# Autodesk Inventor assembly: Assemblage
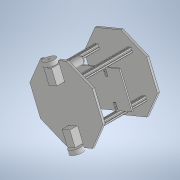
[picture p0: Inventor's stored thumbnail of the model, 180x180]
Saved by Autodesk Inventor 2020 (Build 240168000, 168)
## iProperties
Created: 2019-11-28
Part Number: Assemblage
Document SubType Name: Assembly
Designer: erwan
Author: erwan
## Documents named in this file (7)
- C:\Users\erwan\Desktop\Eirbot\Coupe robotique\Maquette robot\Assemblage.iam
- C:\Users\erwan\Desktop\Eirbot\Coupe robotique\Maquette robot\Pièces\Support bas.ipt
- C:\Users\erwan\Desktop\Eirbot\Coupe robotique\Maquette robot\Pièces\Profilé.ipt
- C:\Users\erwan\Desktop\Eirbot\Coupe robotique\Maquette robot\Pièces\Etage.ipt
- C:\Users\erwan\Desktop\Eirbot\Coupe robotique\Maquette robot\Pièces\Support haut.ipt
- C:\Users\erwan\Desktop\Eirbot\Coupe robotique\Maquette robot\Pièces\Equerre.ipt
- C:\Users\erwan\Desktop\Eirbot\Coupe robotique\Maquette robot\Pièces\Bloc-moteur.ipt
## Components (13 placed, 6 different names)
1. Support bas:1 — Placage:5, Affleurement:1, Affleurement:2, Placage:6, Affleurement:3, Affleurement:4, Placage:7, Placage:8, Placage:9, Placage:10, Affleurement:5, Affleurement:6, Affleurement:7, Affleurement:8, Placage:27, Placage:28, Affleurement:9, Placage:29, Placage:30, Affleurement:10
2. Etage:1 — Placage:5, Affleurement:1, Affleurement:2, Placage:13, Placage:14, Placage:17, Placage:18, Placage:21, Placage:22, Placage:25, Placage:26
3. Support haut:1 — Placage:6, Affleurement:3, Affleurement:4
4. Profilé:1 — Placage:10, Placage:23, Placage:24, Affleurement:8
5. Profilé:2 — Placage:9, Placage:15, Placage:16, Affleurement:6
6. Profilé:3 — Placage:8, Placage:11, Placage:12, Affleurement:5
7. Profilé:4 — Placage:7, Placage:19, Placage:20, Affleurement:7
8. Equerre:1 — Placage:11, Placage:12, Placage:13, Placage:14
9. Equerre:2 — Placage:15, Placage:16, Placage:17, Placage:18
10. Equerre:3 — Placage:19, Placage:20, Placage:21, Placage:22
11. Equerre:4 — Placage:23, Placage:24, Placage:25, Placage:26
12. Bloc-moteur:1 — Placage:29, Placage:30, Affleurement:10
13. Bloc-moteur:2 — Placage:27, Placage:28, Affleurement:9
## Relationships (36: Mate 26, Flush 10)
- Placage:5 [Mate] (125 mm): Support bas:1 ↔ Etage:1
- Affleurement:1 [Flush] (1.5 mm): Support bas:1 ↔ Etage:1
- Affleurement:2 [Flush] (1.5 mm): Support bas:1 ↔ Etage:1
- Placage:6 [Mate] (250 mm): Support bas:1 ↔ Support haut:1
- Affleurement:3 [Flush]: Support bas:1 ↔ Support haut:1
- Affleurement:4 [Flush]: Support bas:1 ↔ Support haut:1
- Placage:7 [Mate]: Support bas:1 ↔ Profilé:4
- Placage:8 [Mate]: Support bas:1 ↔ Profilé:3
- Placage:9 [Mate]: Support bas:1 ↔ Profilé:2
- Placage:10 [Mate]: Support bas:1 ↔ Profilé:1
- Placage:11 [Mate]: Profilé:3 ↔ Equerre:1
- Placage:12 [Mate]: Profilé:3 ↔ Equerre:1
- Placage:13 [Mate]: Etage:1 ↔ Equerre:1
- Placage:14 [Mate]: Etage:1 ↔ Equerre:1
- Placage:15 [Mate]: Profilé:2 ↔ Equerre:2
- Placage:16 [Mate]: Profilé:2 ↔ Equerre:2
- Placage:17 [Mate]: Etage:1 ↔ Equerre:2
- Placage:18 [Mate]: Etage:1 ↔ Equerre:2
- Placage:19 [Mate]: Profilé:4 ↔ Equerre:3
- Placage:20 [Mate]: Profilé:4 ↔ Equerre:3
- Placage:21 [Mate]: Etage:1 ↔ Equerre:3
- Placage:22 [Mate]: Etage:1 ↔ Equerre:3
- Placage:23 [Mate]: Profilé:1 ↔ Equerre:4
- Placage:24 [Mate]: Profilé:1 ↔ Equerre:4
- Placage:25 [Mate]: Etage:1 ↔ Equerre:4
- Placage:26 [Mate]: Etage:1 ↔ Equerre:4
- Affleurement:5 [Flush] (50 mm): Support bas:1 ↔ Profilé:3
- Affleurement:6 [Flush] (50 mm): Support bas:1 ↔ Profilé:2
- Affleurement:7 [Flush] (50 mm): Support bas:1 ↔ Profilé:4
- Affleurement:8 [Flush] (50 mm): Support bas:1 ↔ Profilé:1
- Placage:27 [Mate] (4.9 mm): Support bas:1 ↔ Bloc-moteur:2
- Placage:28 [Mate]: Support bas:1 ↔ Bloc-moteur:2
- Affleurement:9 [Flush] (-10 mm): Support bas:1 ↔ Bloc-moteur:2
- Placage:29 [Mate]: Support bas:1 ↔ Bloc-moteur:1
- Placage:30 [Mate] (4.9 mm): Support bas:1 ↔ Bloc-moteur:1
- Affleurement:10 [Flush] (-10 mm): Support bas:1 ↔ Bloc-moteur:1
